# Autodesk Inventor assembly: AsBuilt Gripper
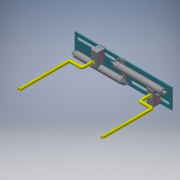
[picture p0: Inventor's stored thumbnail of the model, 180x180]
Saved by Autodesk Inventor 2016 (Build 200138000, 138)
## iProperties
Created: 2015-06-19
Part Number: AsBuilt Gripper
Document SubType Name: Assembly
Designer: steele
Mass: 3030.66 g
Surface Area: 8078.22 cm^2
Volume: 1681.14 cm^3
Density: 1.80274 g/cm^3
Author: steele
## Documents named in this file (13)
- C:\snobotics\CAD-Development\robSteele\SnoBoticsSummer2015\Gripper\AsBuilt Gripper.iam
- C:\snobotics\CAD-MfgResources\McMaster-Carr\Air Cylinder\Pivot Mount Cylinders\Foot Bracket for 1_25 and 1_50 Bore\6498K340.ipt
- C:\snobotics\CAD-Development\robSteele\SnoBoticsSummer2015\Gripper\6498K681.ipt
- C:\snobotics\CAD-Development\robSteele\ipartComponents\ABS Arm.ipt
- C:\snobotics\CAD-Development\robSteele\SnoBoticsSummer2015\Gripper\Gripper Attempt 05\Design Accelerator\Bolted Connection1.iam
- C:\snobotics\CAD-Development\robSteele\SnoBoticsSummer2015\Gripper\Gripper Attempt 05\Design Accelerator\Bolted Connection3.iam
- C:\snobotics\CAD-Development\robSteele\SnoBoticsSummer2015\Gripper\Gripper Attempt 05\Design Accelerator\Bolted Connection4.iam
- C:\snobotics\CAD-Development\robSteele\SnoBoticsSummer2015\Gripper\Gripper Attempt 05\Design Accelerator\Bolted Connection5.iam
- C:\snobotics\CAD-MfgResources\McMaster-Carr\Air Cylinder\Compact Tie Rod Air Cylinder\Square Face\Stroke 2 in\Bore 1 1_16 in\90985A127.ipt
- C:\snobotics\CAD-Development\robSteele\ipartComponents\Aluminum Plate for Gripper\Plate for Gripper 5.5 x 27 x 1(_FS)4 x 3(_FS)8.ipt
- C:\snobotics\CAD-Development\robSteele\ipartComponents\Aluminum Plate for Gripper.ipt
- C:\snobotics\CAD-Development\robSteele\SnoBoticsSummer2015\Gripper\RM Support For Arms With Delrin Slider.ipt
- C:\snobotics\CAD-Development\robSteele\SnoBoticsSummer2015\Gripper\RM Over Support For Arm With Delrin Slider.ipt
## Components (17 placed, 8 different names)
1. Plate for Gripper 5.5 x 27 x 1(_FS)4 x 3(_FS)8:1 — Mate:1, Flush:1, Flush:2, Mate:2, Flush:3, Flush:4, Mate:13, Mate:18, Mate:20, Mate:21
2. 6498K340:1 — Mate:2, Flush:3, Flush:4, Mate:7, Mate:17
3. 6498K340:2 — Mate:1, Flush:1, Flush:2, Mate:8
4. 6498K681:1 — Mate:7
5. 6498K681:2 — Mate:8
6. RM Support For Arms With Delrin Slider:1 — Mate:20, Mate:21, Mate:22, Flush:6
7. RM Support For Arms With Delrin Slider:2 — Mate:13, Mate:19, Flush:5
8. ABS Arm:1 — Insert:6
9. ABS Arm:2 — Insert:5
10. 90985A127:1 — Insert:7
11. 90985A127:2 — Insert:4
12. Bolted Connection:1 [sub-assembly] — Mate:17, Mate:18
13. Bolted Connection:2 [sub-assembly]
14. Bolted Connection:3 [sub-assembly]
15. Bolted Connection:4 [sub-assembly]
16. RM Over Support For Arm With Delrin Slider:1 — Mate:19, Flush:5, Insert:4, Insert:5
17. RM Over Support For Arm With Delrin Slider:2 — Mate:22, Flush:6, Insert:6, Insert:7
## Relationships (21: Mate 11, Flush 6, Insert 4)
- Mate:1: Plate for Gripper 5.5 x 27 x 1(_FS)4 x 3(_FS)8:1 ↔ 6498K340:2
- Flush:1: Plate for Gripper 5.5 x 27 x 1(_FS)4 x 3(_FS)8:1 ↔ 6498K340:2
- Flush:2 (330.2 mm): Plate for Gripper 5.5 x 27 x 1(_FS)4 x 3(_FS)8:1 ↔ 6498K340:2
- Mate:2: Plate for Gripper 5.5 x 27 x 1(_FS)4 x 3(_FS)8:1 ↔ 6498K340:1
- Flush:3: Plate for Gripper 5.5 x 27 x 1(_FS)4 x 3(_FS)8:1 ↔ 6498K340:1
- Flush:4 (330.2 mm): Plate for Gripper 5.5 x 27 x 1(_FS)4 x 3(_FS)8:1 ↔ 6498K340:1
- Mate:7: 6498K340:1 ↔ 6498K681:1
- Mate:8: 6498K340:2 ↔ 6498K681:2
- Mate:13: Plate for Gripper 5.5 x 27 x 1(_FS)4 x 3(_FS)8:1 ↔ RM Support For Arms With Delrin Slider:2
- Mate:17: 6498K340:1 ↔ Bolted Connection:1
- Mate:18: Plate for Gripper 5.5 x 27 x 1(_FS)4 x 3(_FS)8:1 ↔ Bolted Connection:1
- Mate:19: RM Support For Arms With Delrin Slider:2 ↔ RM Over Support For Arm With Delrin Slider:1
- Flush:5: RM Support For Arms With Delrin Slider:2 ↔ RM Over Support For Arm With Delrin Slider:1
- Insert:4: 90985A127:2 ↔ RM Over Support For Arm With Delrin Slider:1
- Mate:20: Plate for Gripper 5.5 x 27 x 1(_FS)4 x 3(_FS)8:1 ↔ RM Support For Arms With Delrin Slider:1
- Mate:21: Plate for Gripper 5.5 x 27 x 1(_FS)4 x 3(_FS)8:1 ↔ RM Support For Arms With Delrin Slider:1
- Mate:22: RM Support For Arms With Delrin Slider:1 ↔ RM Over Support For Arm With Delrin Slider:2
- Flush:6: RM Support For Arms With Delrin Slider:1 ↔ RM Over Support For Arm With Delrin Slider:2
- Insert:5: ABS Arm:2 ↔ RM Over Support For Arm With Delrin Slider:1
- Insert:6: ABS Arm:1 ↔ RM Over Support For Arm With Delrin Slider:2
- Insert:7: 90985A127:1 ↔ RM Over Support For Arm With Delrin Slider:2
## Named parameters: offsetToFrontOfAirCylinder = 330.2 mm
